# Autodesk Inventor assembly: 110033226_iam_13_散步橋
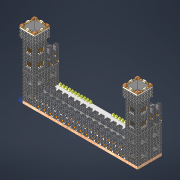
[picture p0: Inventor's stored thumbnail of the model, 180x180]
Saved by Autodesk Inventor 2022 (Build 260153000, 153)
## iProperties
Created: 2022-06-30
Part Number: 110033226_iam_13_散步橋
Document SubType Name: Assembly
Designer: User
Author: User
## Documents named in this file (9)
- D:\D-disk\pomelo\大一\下學期\機械設計製圖\1100332260_LEGOproj_沒有公主城堡\110033226_iam_13_散步橋.iam
- D:\D-disk\pomelo\大一\下學期\機械設計製圖\1100332260_LEGOproj_沒有公主城堡\110033226_ipt_51_散步橋基座.ipt
- D:\D-disk\pomelo\大一\下學期\機械設計製圖\1100332260_LEGOproj_沒有公主城堡\110033226_ipt_28_城堡四圓塔.ipt
- D:\D-disk\pomelo\大一\下學期\機械設計製圖\1100332260_LEGOproj_沒有公主城堡\110033226_iam_06_城堡四角塔.iam
- D:\D-disk\pomelo\大一\下學期\機械設計製圖\1100332260_LEGOproj_沒有公主城堡\110033226_ipt_34_中心城堡圍牆.ipt
- D:\D-disk\pomelo\大一\下學期\機械設計製圖\1100332260_LEGOproj_沒有公主城堡\110033226_ipt_52_散步橋基座二.ipt
- D:\D-disk\pomelo\大一\下學期\機械設計製圖\1100332260_LEGOproj_沒有公主城堡\110033226_ipt_53_散步橋圓柱.ipt
- D:\D-disk\pomelo\大一\下學期\機械設計製圖\1100332260_LEGOproj_沒有公主城堡\110033226_ipt_21_柵欄.ipt
- D:\D-disk\pomelo\大一\下學期\機械設計製圖\1100332260_LEGOproj_沒有公主城堡\110033226_ipt_04_小河.ipt
## Components (117 placed, 8 different names)
1. 110033226_ipt_51_散步橋基座:1 — 貼合:1, 貼合:2, 貼合:3, 貼合:4, 貼合:5, 貼合:6, 貼合:17, 貼合:18, 貼合:19, 貼合:20, 貼合:21, 貼合:22, 貼合:23, 貼合:24, 貼合:25, 貼合:26, 貼合:27, 貼合:28, 貼合:30, 貼合:35, 齊平:1, 貼合:36
2. 110033226_ipt_52_散步橋基座二:1 — 貼合:23, 貼合:24, 貼合:25, 貼合:29, 貼合:31, 貼合:32, 貼合:33
3. 110033226_ipt_21_柵欄:23 — 貼合:32, 貼合:33, 貼合:34
4. 110033226_iam_06_城堡四角塔:1 [sub-assembly] — 貼合:7, 貼合:8, 貼合:9
5. 110033226_iam_06_城堡四角塔:2 [sub-assembly]
6. 110033226_ipt_34_中心城堡圍牆:9 — 貼合:17, 貼合:18, 貼合:19
7. 110033226_ipt_34_中心城堡圍牆:10
8. 110033226_ipt_34_中心城堡圍牆:11
9. 110033226_ipt_34_中心城堡圍牆:12
10. 110033226_ipt_34_中心城堡圍牆:13
11. 110033226_ipt_34_中心城堡圍牆:14
12. 110033226_ipt_34_中心城堡圍牆:15
13. 110033226_ipt_34_中心城堡圍牆:16
14. 110033226_ipt_34_中心城堡圍牆:17
15. 110033226_ipt_34_中心城堡圍牆:18
16. 110033226_ipt_34_中心城堡圍牆:19
17. 110033226_ipt_34_中心城堡圍牆:20
18. 110033226_ipt_34_中心城堡圍牆:21
19. 110033226_ipt_34_中心城堡圍牆:22
20. 110033226_ipt_34_中心城堡圍牆:23
21. 110033226_ipt_34_中心城堡圍牆:24 — 貼合:20, 貼合:21, 貼合:22
22. 110033226_ipt_34_中心城堡圍牆:25
23. 110033226_ipt_34_中心城堡圍牆:26
24. 110033226_ipt_34_中心城堡圍牆:27
25. 110033226_ipt_34_中心城堡圍牆:28
26. 110033226_ipt_34_中心城堡圍牆:29
27. 110033226_ipt_34_中心城堡圍牆:30
28. 110033226_ipt_34_中心城堡圍牆:31
29. 110033226_ipt_34_中心城堡圍牆:32
30. 110033226_ipt_34_中心城堡圍牆:33
31. 110033226_ipt_34_中心城堡圍牆:34
32. 110033226_ipt_34_中心城堡圍牆:35
33. 110033226_ipt_34_中心城堡圍牆:36
34. 110033226_ipt_34_中心城堡圍牆:37
35. 110033226_ipt_34_中心城堡圍牆:38
36. 110033226_ipt_53_散步橋圓柱:1 — 貼合:26, 貼合:27, 貼合:28
37. 110033226_ipt_53_散步橋圓柱:4
38. 110033226_ipt_53_散步橋圓柱:5
39. 110033226_ipt_53_散步橋圓柱:6
40. 110033226_ipt_53_散步橋圓柱:7
41. 110033226_ipt_53_散步橋圓柱:8
42. 110033226_ipt_53_散步橋圓柱:9
43. 110033226_ipt_53_散步橋圓柱:10
44. 110033226_ipt_53_散步橋圓柱:11
45. 110033226_ipt_53_散步橋圓柱:12
46. 110033226_ipt_53_散步橋圓柱:13
47. 110033226_ipt_53_散步橋圓柱:14
48. 110033226_ipt_53_散步橋圓柱:15
49. 110033226_ipt_53_散步橋圓柱:16
50. 110033226_ipt_53_散步橋圓柱:17
51. 110033226_ipt_53_散步橋圓柱:18
52. 110033226_ipt_53_散步橋圓柱:19
53. 110033226_ipt_53_散步橋圓柱:20
54. 110033226_ipt_53_散步橋圓柱:21
55. 110033226_ipt_53_散步橋圓柱:22
56. 110033226_ipt_53_散步橋圓柱:23
57. 110033226_ipt_53_散步橋圓柱:24
58. 110033226_ipt_53_散步橋圓柱:25
59. 110033226_ipt_53_散步橋圓柱:26
60. 110033226_ipt_04_小河:1 — 貼合:35, 齊平:1, 貼合:36
61. 110033226_ipt_04_小河:2
62. 110033226_ipt_04_小河:3
63. 110033226_ipt_04_小河:4
64. 110033226_ipt_04_小河:5
65. 110033226_ipt_04_小河:6
66. 110033226_ipt_04_小河:7
67. 110033226_ipt_04_小河:8
68. 110033226_ipt_04_小河:9
69. 110033226_ipt_04_小河:10
70. 110033226_ipt_04_小河:11
71. 110033226_ipt_04_小河:12
72. 110033226_ipt_04_小河:13
73. 110033226_ipt_04_小河:14
74. 110033226_ipt_04_小河:15
75. 110033226_ipt_04_小河:16
76. 110033226_ipt_04_小河:17
77. 110033226_ipt_04_小河:18
78. 110033226_ipt_04_小河:19
79. 110033226_ipt_04_小河:20
80. 110033226_ipt_04_小河:21
81. 110033226_ipt_04_小河:22
82. 110033226_ipt_04_小河:23
83. 110033226_ipt_04_小河:24
84. 110033226_ipt_28_城堡四圓塔:1 — 貼合:4, 貼合:5, 貼合:6, 貼合:7, 貼合:10, 貼合:11, 貼合:12, 貼合:13, 貼合:14, 貼合:15, 貼合:16
85. 110033226_ipt_28_城堡四圓塔:2 — 貼合:8, 貼合:9
86. 110033226_ipt_28_城堡四圓塔:3
87. 110033226_ipt_28_城堡四圓塔:4
88. 110033226_ipt_34_中心城堡圍牆:1 — 貼合:10, 貼合:11, 貼合:12, 貼合:13
89. 110033226_ipt_34_中心城堡圍牆:3
90. 110033226_ipt_34_中心城堡圍牆:2 — 貼合:14, 貼合:15, 貼合:16
91. 110033226_ipt_34_中心城堡圍牆:4
92. 110033226_ipt_34_中心城堡圍牆:5
93. 110033226_ipt_34_中心城堡圍牆:6
94. 110033226_ipt_34_中心城堡圍牆:7
95. 110033226_ipt_34_中心城堡圍牆:8
96. 110033226_ipt_21_柵欄:1 — 貼合:29, 貼合:30, 貼合:31
97. 110033226_ipt_21_柵欄:2
98. 110033226_ipt_21_柵欄:3
99. 110033226_ipt_21_柵欄:4
100. 110033226_ipt_21_柵欄:5
101. 110033226_ipt_21_柵欄:6
102. 110033226_ipt_21_柵欄:7
103. 110033226_ipt_21_柵欄:8
104. 110033226_ipt_21_柵欄:9
105. 110033226_ipt_21_柵欄:10
106. 110033226_ipt_21_柵欄:11
107. 110033226_ipt_21_柵欄:12
108. 110033226_ipt_21_柵欄:13
109. 110033226_ipt_21_柵欄:14
110. 110033226_ipt_21_柵欄:15
111. 110033226_ipt_21_柵欄:16
112. 110033226_ipt_21_柵欄:17
113. 110033226_ipt_21_柵欄:18
114. 110033226_ipt_21_柵欄:19
115. 110033226_ipt_21_柵欄:20
116. 110033226_ipt_21_柵欄:21
117. 110033226_ipt_21_柵欄:22 — 貼合:34
## Component patterns: (2 elements), (2 elements, first: 110033226_iam_06_城堡四角塔:1), (2 elements), (15 elements, first: 110033226_ipt_34_中心城堡圍牆:9), (15 elements, first: 110033226_ipt_34_中心城堡圍牆:24), (24 elements, first: 110033226_ipt_53_散步橋圓柱:1), (2 elements), (24 elements, first: 110033226_ipt_04_小河:1), (2 elements, first: 110033226_ipt_28_城堡四圓塔:1), 元件陣列 1:2 (2 elements), (2 elements, first: 110033226_ipt_34_中心城堡圍牆:1), (2 elements, first: 110033226_ipt_34_中心城堡圍牆:2), 元件陣列 4:2 (2 elements), 元件陣列 5:2 (2 elements), (11 elements, first: 110033226_ipt_21_柵欄:1), 元件陣列 10:2 (11 elements)
## Relationships (37: Mate 36, Flush 1)
- 貼合:1 [Mate]: 110033226_ipt_51_散步橋基座:1
- 貼合:2 [Mate]: 110033226_ipt_51_散步橋基座:1
- 貼合:3 [Mate]: 110033226_ipt_51_散步橋基座:1
- 貼合:4 [Mate]: 110033226_ipt_51_散步橋基座:1 ↔ 110033226_ipt_28_城堡四圓塔:1
- 貼合:5 [Mate]: 110033226_ipt_51_散步橋基座:1 ↔ 110033226_ipt_28_城堡四圓塔:1
- 貼合:6 [Mate]: 110033226_ipt_51_散步橋基座:1 ↔ 110033226_ipt_28_城堡四圓塔:1
- 貼合:7 [Mate]: 110033226_iam_06_城堡四角塔:1 ↔ 110033226_ipt_28_城堡四圓塔:1
- 貼合:8 [Mate]: 110033226_iam_06_城堡四角塔:1 ↔ 110033226_ipt_28_城堡四圓塔:2
- 貼合:9 [Mate]: 110033226_iam_06_城堡四角塔:1 ↔ 110033226_ipt_28_城堡四圓塔:2
- 貼合:10 [Mate]: 110033226_ipt_28_城堡四圓塔:1 ↔ 110033226_ipt_34_中心城堡圍牆:1
- 貼合:11 [Mate]: 110033226_ipt_28_城堡四圓塔:1 ↔ 110033226_ipt_34_中心城堡圍牆:1
- 貼合:12 [Mate]: 110033226_ipt_28_城堡四圓塔:1 ↔ 110033226_ipt_34_中心城堡圍牆:1
- 貼合:13 [Mate]: 110033226_ipt_28_城堡四圓塔:1 ↔ 110033226_ipt_34_中心城堡圍牆:1
- 貼合:14 [Mate]: 110033226_ipt_28_城堡四圓塔:1 ↔ 110033226_ipt_34_中心城堡圍牆:2
- 貼合:15 [Mate]: 110033226_ipt_28_城堡四圓塔:1 ↔ 110033226_ipt_34_中心城堡圍牆:2
- 貼合:16 [Mate]: 110033226_ipt_28_城堡四圓塔:1 ↔ 110033226_ipt_34_中心城堡圍牆:2
- 貼合:17 [Mate]: 110033226_ipt_51_散步橋基座:1 ↔ 110033226_ipt_34_中心城堡圍牆:9
- 貼合:18 [Mate]: 110033226_ipt_51_散步橋基座:1 ↔ 110033226_ipt_34_中心城堡圍牆:9
- 貼合:19 [Mate]: 110033226_ipt_51_散步橋基座:1 ↔ 110033226_ipt_34_中心城堡圍牆:9
- 貼合:20 [Mate]: 110033226_ipt_51_散步橋基座:1 ↔ 110033226_ipt_34_中心城堡圍牆:24
- 貼合:21 [Mate]: 110033226_ipt_51_散步橋基座:1 ↔ 110033226_ipt_34_中心城堡圍牆:24
- 貼合:22 [Mate]: 110033226_ipt_51_散步橋基座:1 ↔ 110033226_ipt_34_中心城堡圍牆:24
- 貼合:23 [Mate] (23.5 mm): 110033226_ipt_51_散步橋基座:1 ↔ 110033226_ipt_52_散步橋基座二:1
- 貼合:24 [Mate]: 110033226_ipt_51_散步橋基座:1 ↔ 110033226_ipt_52_散步橋基座二:1
- 貼合:25 [Mate]: 110033226_ipt_51_散步橋基座:1 ↔ 110033226_ipt_52_散步橋基座二:1
- 貼合:26 [Mate]: 110033226_ipt_51_散步橋基座:1 ↔ 110033226_ipt_53_散步橋圓柱:1
- 貼合:27 [Mate]: 110033226_ipt_51_散步橋基座:1 ↔ 110033226_ipt_53_散步橋圓柱:1
- 貼合:28 [Mate]: 110033226_ipt_51_散步橋基座:1 ↔ 110033226_ipt_53_散步橋圓柱:1
- 貼合:29 [Mate]: 110033226_ipt_52_散步橋基座二:1 ↔ 110033226_ipt_21_柵欄:1
- 貼合:30 [Mate]: 110033226_ipt_51_散步橋基座:1 ↔ 110033226_ipt_21_柵欄:1
- 貼合:31 [Mate]: 110033226_ipt_52_散步橋基座二:1 ↔ 110033226_ipt_21_柵欄:1
- 貼合:32 [Mate]: 110033226_ipt_52_散步橋基座二:1 ↔ 110033226_ipt_21_柵欄:23
- 貼合:33 [Mate]: 110033226_ipt_52_散步橋基座二:1 ↔ 110033226_ipt_21_柵欄:23
- 貼合:34 [Mate]: 110033226_ipt_21_柵欄:23 ↔ 110033226_ipt_21_柵欄:22
- 貼合:35 [Mate]: 110033226_ipt_51_散步橋基座:1 ↔ 110033226_ipt_04_小河:1
- 齊平:1 [Flush]: 110033226_ipt_51_散步橋基座:1 ↔ 110033226_ipt_04_小河:1
- 貼合:36 [Mate]: 110033226_ipt_51_散步橋基座:1 ↔ 110033226_ipt_04_小河:1
